# Autodesk Inventor assembly: CartesianRobotWorkSpace
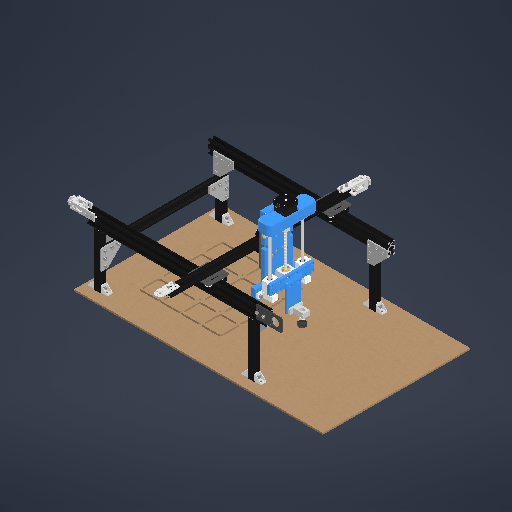
[picture p0: Inventor's stored thumbnail of the model, 512x512]
Saved by Autodesk Inventor 2027.1 (Build 311270010, 270A)
## iProperties
Created: 2026-09-29
Part Number: CartesianRobotWorkSpace
Document SubType Name: Assembly
Designer: SDS Scholar
Author: SDS Scholar
## Documents named in this file (18)
- E:\Apps\AutodeskInventor\University\MCT333_Design_of_Mechatronics_Systems_1\CAD\cartesian_robot_workspace\CartesianRobotWorkSpace.iam
- E:\Apps\AutodeskInventor\University\MCT333_Design_of_Mechatronics_Systems_1\CAD\cartesian_robot_workspace\UpperBase.ipt
- E:\Apps\AutodeskInventor\University\MCT333_Design_of_Mechatronics_Systems_1\CAD\cartesian_robot_workspace\ProductsStoringGrid.ipt
- E:\Apps\AutodeskInventor\University\MCT333_Design_of_Mechatronics_Systems_1\CAD\off_the_shelf_components\AluminiumExtrusion\AluminiumExtrusion2020\Pillars.ipt
- E:\Apps\AutodeskInventor\University\MCT333_Design_of_Mechatronics_Systems_1\CAD\off_the_shelf_components\CornerBracket2020\CornerBracket2020.ipt
- C:\Users\SDS Scholar\Documents\Inventor\Content Center Files\R2027\en-US\SS-ISO 4762\ISO 4762 - M5 x 10SS-ISO.ipt
- E:\Apps\AutodeskInventor\University\MCT333_Design_of_Mechatronics_Systems_1\CAD\off_the_shelf_components\T_nuts\Slider T-Nut for 2020 - M5.ipt
- E:\Apps\AutodeskInventor\University\MCT333_Design_of_Mechatronics_Systems_1\CAD\off_the_shelf_components\RightAngleCornerPlate2020\2020 corner joining plate v1.ipt
- E:\Apps\AutodeskInventor\University\MCT333_Design_of_Mechatronics_Systems_1\CAD\off_the_shelf_components\AluminiumExtrusion\Extrusion2040\2040extrusion_ipt\X_Axis.ipt
- E:\Apps\AutodeskInventor\University\MCT333_Design_of_Mechatronics_Systems_1\CAD\off_the_shelf_components\AluminiumExtrusion\AluminiumExtrusion2020\SupportBeam.ipt
- E:\Apps\AutodeskInventor\University\MCT333_Design_of_Mechatronics_Systems_1\CAD\off_the_shelf_components\VSoltGantrySetAllSizes\20mm Gantry Set\20mm Gantry Set.ipt
- E:\Apps\AutodeskInventor\University\MCT333_Design_of_Mechatronics_Systems_1\CAD\off_the_shelf_components\RightAngleCornerPlate2020\2020 corner joining plate v1_MIR2.ipt
- E:\Apps\AutodeskInventor\University\MCT333_Design_of_Mechatronics_Systems_1\CAD\off_the_shelf_components\T_nuts\Slider T-Nut for 2020 - M5_MIR2.ipt
- E:\Apps\AutodeskInventor\University\MCT333_Design_of_Mechatronics_Systems_1\CAD\off_the_shelf_components\nema-17-23-stepper-motor-mounts\NEMA 17 Flat.ipt
- E:\Apps\AutodeskInventor\University\MCT333_Design_of_Mechatronics_Systems_1\CAD\off_the_shelf_components\GT2BeltTensioner\2020 Belt Tensioner G_K.ipt
- E:\Apps\AutodeskInventor\University\MCT333_Design_of_Mechatronics_Systems_1\CAD\cartesian_robot_workspace\Y_Axis.iam
- E:\Apps\AutodeskInventor\University\MCT333_Design_of_Mechatronics_Systems_1\CAD\cartesian_robot_workspace\Z Axis\Z-Axis.iam
- E:\Apps\AutodeskInventor\University\MCT333_Design_of_Mechatronics_Systems_1\CAD\DESIGN1_CAD_parameters.xlsx
## Components (118 placed, 16 different names)
1. UpperBase:1 — Mate:1, Mate:2, Flush:1, Mate:4, Mate:5, Mate:6, Mate:7, Mate:8, Mate:9, Mate:10, Mate:11, Mate:12, Mate:15, Flush:2, Mate:16, Mate:17, Mate:26, Mate:27
2. ProductsStoringGrid:1 — Mate:4, Mate:5, Mate:6, Mate:7
3. ProductsStoringGrid:2 — Mate:8, Mate:9, Mate:10, Mate:11
4. Z-Axis:1 [sub-assembly] — Tangent:9, Tangent:10, Tangent:11, Tangent:12
5. SupportBeam:1 — Mate:88, Mate:123, Mate:124, Mate:125, Mate:126, Mate:138, Mate:141, Mate:143
6. X_Axis:1 — Mate:32, Mate:33, Mate:34, Mate:35, Mate:36, Mate:37, Mate:48, Mate:49, Mate:56, Mate:59, Flush:3, Mate:60, Tangent:1, Tangent:2, Tangent:3, Tangent:4, Mate:145, Mate:146, Mate:147, Mate:148, Mate:151, Mate:154, Mate:155, Flush:6, Mate:156, Mate:157, Mate:158, Mate:159, Mate:162, Mate:165, Flush:7, Mate:182
7. X_Axis:2 — Mate:89, Mate:90, Mate:91, Mate:92, Mate:93, Mate:94, Mate:107, Mate:110, Mate:113, Mate:115, Flush:4, Mate:116, Tangent:5, Tangent:6, Tangent:7, Tangent:8
8. NEMA 17 Flat:1 — Mate:149, Mate:152, Mate:155
9. Slider T-Nut for 2020 - M5:40 — Mate:145, Mate:146, Mate:150, Flush:6
10. Slider T-Nut for 2020 - M5:41 — Mate:147, Mate:148, Mate:153
11. SS ISO 4762 M5 x 10:58 — Mate:149, Mate:150, Mate:151
12. SS ISO 4762 M5 x 10:59 — Mate:152, Mate:153, Mate:154
13. 2020 Belt Tensioner G_K:1 — Mate:180, Mate:181, Mate:182
14. SS ISO 4762 M5 x 10:60 — Mate:164, Mate:165, Mate:181
15. SS ISO 4762 M5 x 10:61 — Mate:161, Mate:162, Mate:179, Mate:180
16. Slider T-Nut for 2020 - M5:42 — Mate:156, Mate:157, Mate:161, Mate:179
17. Slider T-Nut for 2020 - M5:43 — Mate:158, Mate:159, Mate:164, Flush:7
18. 20mm Gantry Set:1 — Tangent:1, Tangent:2, Tangent:3, Tangent:4, Flush:5, Mate:171, Flush:9
19. 20mm Gantry Set:2 — Tangent:5, Tangent:6, Tangent:7, Tangent:8, Flush:5, Mate:174, Mate:177, Flush:8, Flush:9
20. Y_Axis:1 [sub-assembly] — Mate:167, Mate:168, Mate:169, Mate:170, Mate:173, Mate:176, Mate:177, Flush:8, Tangent:9, Tangent:10, Tangent:11, Tangent:12
21. Slider T-Nut for 2020 - M5:44 — Mate:167, Mate:168, Mate:172
22. Slider T-Nut for 2020 - M5:45 — Mate:169, Mate:170, Mate:175
23. SS ISO 4762 M5 x 10:62 — Mate:174, Mate:175, Mate:176
24. SS ISO 4762 M5 x 10:63 — Mate:171, Mate:172, Mate:173
25. Pillars:1 — Flush:2, Mate:18, Mate:19, Mate:22, Mate:24, Mate:25, Mate:30, Mate:88, Mate:117, Mate:118, Mate:119, Mate:120, Mate:121, Mate:122, Mate:129, Mate:132, Mate:135, Mate:142, Symmetry:1
26. CornerBracket2020:4 — Mate:15, Mate:26, Mate:27, Mate:28
27. CornerBracket2020:1 — Mate:12, Mate:16, Mate:17, Mate:20, Mate:31
28. SS ISO 4762 M5 x 10:1 — Mate:20, Mate:21, Mate:22, Mate:31
29. Slider T-Nut for 2020 - M5:1 — Mate:18, Mate:19, Mate:21
30. Slider T-Nut for 2020 - M5:2 — Mate:24, Mate:25, Mate:29
31. SS ISO 4762 M5 x 10:2 — Mate:28, Mate:29, Mate:30
32. Pillars:2 — Mate:95, Mate:96, Mate:97, Mate:98, Mate:101, Mate:104, Mate:114, Mate:116
33. CornerBracket2020:5
34. CornerBracket2020:6
35. SS ISO 4762 M5 x 10:3
36. Slider T-Nut for 2020 - M5:3
37. Slider T-Nut for 2020 - M5:4
38. SS ISO 4762 M5 x 10:4
39. Pillars:3 — Symmetry:1
40. CornerBracket2020:7
41. CornerBracket2020:8
42. SS ISO 4762 M5 x 10:5
43. Slider T-Nut for 2020 - M5:5
44. Slider T-Nut for 2020 - M5:6
45. SS ISO 4762 M5 x 10:6
46. Pillars:4 — Mate:38, Mate:39, Mate:40, Mate:41, Mate:44, Mate:45, Mate:53, Mate:60
47. CornerBracket2020:9
48. CornerBracket2020:10
49. SS ISO 4762 M5 x 10:7
50. Slider T-Nut for 2020 - M5:7
51. Slider T-Nut for 2020 - M5:8
52. SS ISO 4762 M5 x 10:8
53. 2020 corner joining plate v1:6 — Mate:127, Mate:130, Mate:133, Mate:136, Mate:139, Mate:142, Mate:143, Mate:144
54. Slider T-Nut for 2020 - M5:35 — Mate:119, Mate:120, Mate:131
55. Slider T-Nut for 2020 - M5:36 — Mate:123, Mate:124, Mate:137
56. Slider T-Nut for 2020 - M5:37 — Mate:117, Mate:118, Mate:134
57. Slider T-Nut for 2020 - M5:38 — Mate:125, Mate:126, Mate:140
58. Slider T-Nut for 2020 - M5:39 — Mate:121, Mate:122, Mate:128
59. SS ISO 4762 M5 x 10:48 — Mate:127, Mate:128, Mate:129
60. SS ISO 4762 M5 x 10:49 — Mate:139, Mate:140, Mate:141
61. SS ISO 4762 M5 x 10:50 — Mate:130, Mate:131, Mate:132
62. SS ISO 4762 M5 x 10:51 — Mate:133, Mate:134, Mate:135
63. SS ISO 4762 M5 x 10:52 — Mate:136, Mate:137, Mate:138
64. 2020 corner joining plate v1_MIR2:1
65. Slider T-Nut for 2020 - M5_MIR2:1
66. Slider T-Nut for 2020 - M5_MIR2:2
67. Slider T-Nut for 2020 - M5_MIR2:3
68. Slider T-Nut for 2020 - M5_MIR2:4
69. Slider T-Nut for 2020 - M5_MIR2:5
70. SS ISO 4762 M5 x 10:53
71. SS ISO 4762 M5 x 10:54
72. SS ISO 4762 M5 x 10:55
73. SS ISO 4762 M5 x 10:56
74. SS ISO 4762 M5 x 10:57
75. 2020 corner joining plate v1:1 — Mate:42, Mate:45, Mate:46, Mate:49, Mate:51, Mate:54, Mate:57, Flush:3
76. Slider T-Nut for 2020 - M5:9 — Mate:36, Mate:37, Mate:55
77. Slider T-Nut for 2020 - M5:10 — Mate:38, Mate:39, Mate:52
78. Slider T-Nut for 2020 - M5:11 — Mate:40, Mate:41, Mate:43
79. Slider T-Nut for 2020 - M5:12 — Mate:34, Mate:35, Mate:58
80. Slider T-Nut for 2020 - M5:13 — Mate:32, Mate:33, Mate:47
81. SS ISO 4762 M5 x 10:9 — Mate:42, Mate:43, Mate:44
82. SS ISO 4762 M5 x 10:10 — Mate:46, Mate:47, Mate:48
83. SS ISO 4762 M5 x 10:11 — Mate:54, Mate:55, Mate:56
84. SS ISO 4762 M5 x 10:12 — Mate:51, Mate:52, Mate:53
85. SS ISO 4762 M5 x 10:13 — Mate:57, Mate:58, Mate:59
86. 2020 corner joining plate v1:2
87. Slider T-Nut for 2020 - M5:14
88. Slider T-Nut for 2020 - M5:15
89. Slider T-Nut for 2020 - M5:16
90. Slider T-Nut for 2020 - M5:17
91. Slider T-Nut for 2020 - M5:18
92. SS ISO 4762 M5 x 10:14
93. SS ISO 4762 M5 x 10:15
94. SS ISO 4762 M5 x 10:16
95. SS ISO 4762 M5 x 10:17
96. SS ISO 4762 M5 x 10:18
97. 2020 corner joining plate v1:4 — Mate:99, Mate:102, Mate:105, Mate:108, Mate:111, Mate:114, Mate:115, Flush:4
98. Slider T-Nut for 2020 - M5:25 — Mate:93, Mate:94, Mate:106
99. Slider T-Nut for 2020 - M5:26 — Mate:95, Mate:96, Mate:103
100. Slider T-Nut for 2020 - M5:27 — Mate:97, Mate:98, Mate:100
101. Slider T-Nut for 2020 - M5:28 — Mate:91, Mate:92, Mate:109
102. Slider T-Nut for 2020 - M5:29 — Mate:89, Mate:90, Mate:112
103. SS ISO 4762 M5 x 10:38 — Mate:99, Mate:100, Mate:101
104. SS ISO 4762 M5 x 10:39 — Mate:105, Mate:106, Mate:107
105. SS ISO 4762 M5 x 10:40 — Mate:102, Mate:103, Mate:104
106. SS ISO 4762 M5 x 10:41 — Mate:108, Mate:109, Mate:110
107. SS ISO 4762 M5 x 10:42 — Mate:111, Mate:112, Mate:113
108. 2020 corner joining plate v1:5 — Mate:144
109. Slider T-Nut for 2020 - M5:30
110. Slider T-Nut for 2020 - M5:31
111. Slider T-Nut for 2020 - M5:32
112. Slider T-Nut for 2020 - M5:33
113. Slider T-Nut for 2020 - M5:34
114. SS ISO 4762 M5 x 10:43
115. SS ISO 4762 M5 x 10:44
116. SS ISO 4762 M5 x 10:45
117. SS ISO 4762 M5 x 10:46
118. SS ISO 4762 M5 x 10:47
## Component patterns: (4 elements, first: Pillars:1 + CornerBracket2020:4 + CornerBracket2020:1 + SS ISO 4762 M5 x 10:1 + Slider T-Nut for 2020 - M5:1 + Slider T-Nut for 2020 - M5:2 + SS ISO 4762 M5 x 10:2), (2 elements, first: 2020 corner joining plate v1:6 + Slider T-Nut for 2020 - M5:35 + Slider T-Nut for 2020 - M5:36 + Slider T-Nut for 2020 - M5:37 + Slider T-Nut for 2020 - M5:38 + Slider T-Nut for 2020 - M5:39 + SS ISO 4762 M5 x 10:48 + SS ISO 4762 M5 x 10:49 + SS ISO 4762 M5 x 10:50 + SS ISO 4762 M5 x 10:51 + SS ISO 4762 M5 x 10:52), (2 elements, first: 2020 corner joining plate v1:1 + Slider T-Nut for 2020 - M5:9 + Slider T-Nut for 2020 - M5:10 + Slider T-Nut for 2020 - M5:11 + Slider T-Nut for 2020 - M5:12 + Slider T-Nut for 2020 - M5:13 + SS ISO 4762 M5 x 10:9 + SS ISO 4762 M5 x 10:10 + SS ISO 4762 M5 x 10:11 + SS ISO 4762 M5 x 10:12 + SS ISO 4762 M5 x 10:13), (2 elements, first: 2020 corner joining plate v1:4 + Slider T-Nut for 2020 - M5:25 + Slider T-Nut for 2020 - M5:26 + Slider T-Nut for 2020 - M5:27 + Slider T-Nut for 2020 - M5:28 + Slider T-Nut for 2020 - M5:29 + SS ISO 4762 M5 x 10:38 + SS ISO 4762 M5 x 10:39 + SS ISO 4762 M5 x 10:40 + SS ISO 4762 M5 x 10:41 + SS ISO 4762 M5 x 10:42)
## Relationships (168: Mate 146, Tangent 12, Flush 9, Symmetry 1)
- Mate:1: UpperBase:1
- Mate:2: UpperBase:1
- Flush:1: UpperBase:1
- Mate:4: UpperBase:1 ↔ ProductsStoringGrid:1
- Mate:5: UpperBase:1 ↔ ProductsStoringGrid:1
- Mate:6: UpperBase:1 ↔ ProductsStoringGrid:1
- Mate:7: UpperBase:1 ↔ ProductsStoringGrid:1
- Mate:8: UpperBase:1 ↔ ProductsStoringGrid:2
- Mate:9: UpperBase:1 ↔ ProductsStoringGrid:2
- Mate:10: UpperBase:1 ↔ ProductsStoringGrid:2
- Mate:11: UpperBase:1 ↔ ProductsStoringGrid:2
- Mate:12: UpperBase:1 ↔ CornerBracket2020:1
- Mate:15: UpperBase:1 ↔ CornerBracket2020:4
- Flush:2: UpperBase:1 ↔ Pillars:1
- Mate:16: UpperBase:1 ↔ CornerBracket2020:1
- Mate:17: UpperBase:1 ↔ CornerBracket2020:1
- Mate:18: Pillars:1 ↔ Slider T-Nut for 2020 - M5:1
- Mate:19: Pillars:1 ↔ Slider T-Nut for 2020 - M5:1
- Mate:20: CornerBracket2020:1 ↔ SS ISO 4762 M5 x 10:1
- Mate:21: SS ISO 4762 M5 x 10:1 ↔ Slider T-Nut for 2020 - M5:1
- Mate:22: Pillars:1 ↔ SS ISO 4762 M5 x 10:1
- Mate:24: Pillars:1 ↔ Slider T-Nut for 2020 - M5:2
- Mate:25: Pillars:1 ↔ Slider T-Nut for 2020 - M5:2
- Mate:26: UpperBase:1 ↔ CornerBracket2020:4
- Mate:27: UpperBase:1 ↔ CornerBracket2020:4
- Mate:28: CornerBracket2020:4 ↔ SS ISO 4762 M5 x 10:2
- Mate:29: Slider T-Nut for 2020 - M5:2 ↔ SS ISO 4762 M5 x 10:2
- Mate:30: Pillars:1 ↔ SS ISO 4762 M5 x 10:2
- Mate:31 (0.7 mm): CornerBracket2020:1 ↔ SS ISO 4762 M5 x 10:1
- Mate:32: X_Axis:1 ↔ Slider T-Nut for 2020 - M5:13
- Mate:33: X_Axis:1 ↔ Slider T-Nut for 2020 - M5:13
- Mate:34: X_Axis:1 ↔ Slider T-Nut for 2020 - M5:12
- Mate:35: X_Axis:1 ↔ Slider T-Nut for 2020 - M5:12
- Mate:36: X_Axis:1 ↔ Slider T-Nut for 2020 - M5:9
- Mate:37: X_Axis:1 ↔ Slider T-Nut for 2020 - M5:9
- Mate:38: Pillars:4 ↔ Slider T-Nut for 2020 - M5:10
- Mate:39: Pillars:4 ↔ Slider T-Nut for 2020 - M5:10
- Mate:40: Pillars:4 ↔ Slider T-Nut for 2020 - M5:11
- Mate:41: Pillars:4 ↔ Slider T-Nut for 2020 - M5:11
- Mate:42: 2020 corner joining plate v1:1 ↔ SS ISO 4762 M5 x 10:9
- Mate:43: Slider T-Nut for 2020 - M5:11 ↔ SS ISO 4762 M5 x 10:9
- Mate:44: Pillars:4 ↔ SS ISO 4762 M5 x 10:9
- Mate:45: Pillars:4 ↔ 2020 corner joining plate v1:1
- Mate:46: 2020 corner joining plate v1:1 ↔ SS ISO 4762 M5 x 10:10
- Mate:47: Slider T-Nut for 2020 - M5:13 ↔ SS ISO 4762 M5 x 10:10
- Mate:48: X_Axis:1 ↔ SS ISO 4762 M5 x 10:10
- Mate:49: X_Axis:1 ↔ 2020 corner joining plate v1:1
- Mate:51: 2020 corner joining plate v1:1 ↔ SS ISO 4762 M5 x 10:12
- Mate:52: Slider T-Nut for 2020 - M5:10 ↔ SS ISO 4762 M5 x 10:12
- Mate:53: Pillars:4 ↔ SS ISO 4762 M5 x 10:12
- Mate:54: 2020 corner joining plate v1:1 ↔ SS ISO 4762 M5 x 10:11
- Mate:55: Slider T-Nut for 2020 - M5:9 ↔ SS ISO 4762 M5 x 10:11
- Mate:56: X_Axis:1 ↔ SS ISO 4762 M5 x 10:11
- Mate:57: 2020 corner joining plate v1:1 ↔ SS ISO 4762 M5 x 10:13
- Mate:58: Slider T-Nut for 2020 - M5:12 ↔ SS ISO 4762 M5 x 10:13
- Mate:59: X_Axis:1 ↔ SS ISO 4762 M5 x 10:13
- Flush:3: X_Axis:1 ↔ 2020 corner joining plate v1:1
- Mate:60: X_Axis:1 ↔ Pillars:4
- Mate:88: SupportBeam:1 ↔ Pillars:1
- Tangent:1: X_Axis:1 ↔ 20mm Gantry Set:1
- Tangent:2: X_Axis:1 ↔ 20mm Gantry Set:1
- Tangent:3: X_Axis:1 ↔ 20mm Gantry Set:1
- Tangent:4: X_Axis:1 ↔ 20mm Gantry Set:1
- Mate:89: X_Axis:2 ↔ Slider T-Nut for 2020 - M5:29
- Mate:90: X_Axis:2 ↔ Slider T-Nut for 2020 - M5:29
- Mate:91: X_Axis:2 ↔ Slider T-Nut for 2020 - M5:28
- Mate:92: X_Axis:2 ↔ Slider T-Nut for 2020 - M5:28
- Mate:93: X_Axis:2 ↔ Slider T-Nut for 2020 - M5:25
- Mate:94: X_Axis:2 ↔ Slider T-Nut for 2020 - M5:25
- Mate:95: Pillars:2 ↔ Slider T-Nut for 2020 - M5:26
- Mate:96: Pillars:2 ↔ Slider T-Nut for 2020 - M5:26
- Mate:97: Pillars:2 ↔ Slider T-Nut for 2020 - M5:27
- Mate:98: Pillars:2 ↔ Slider T-Nut for 2020 - M5:27
- Mate:99: 2020 corner joining plate v1:4 ↔ SS ISO 4762 M5 x 10:38
- Mate:100: Slider T-Nut for 2020 - M5:27 ↔ SS ISO 4762 M5 x 10:38
- Mate:101: Pillars:2 ↔ SS ISO 4762 M5 x 10:38
- Mate:102: 2020 corner joining plate v1:4 ↔ SS ISO 4762 M5 x 10:40
- Mate:103: Slider T-Nut for 2020 - M5:26 ↔ SS ISO 4762 M5 x 10:40
- Mate:104: Pillars:2 ↔ SS ISO 4762 M5 x 10:40
- Mate:105: 2020 corner joining plate v1:4 ↔ SS ISO 4762 M5 x 10:39
- Mate:106: Slider T-Nut for 2020 - M5:25 ↔ SS ISO 4762 M5 x 10:39
- Mate:107: X_Axis:2 ↔ SS ISO 4762 M5 x 10:39
- Mate:108: 2020 corner joining plate v1:4 ↔ SS ISO 4762 M5 x 10:41
- Mate:109: Slider T-Nut for 2020 - M5:28 ↔ SS ISO 4762 M5 x 10:41
- Mate:110: X_Axis:2 ↔ SS ISO 4762 M5 x 10:41
- Mate:111: 2020 corner joining plate v1:4 ↔ SS ISO 4762 M5 x 10:42
- Mate:112: Slider T-Nut for 2020 - M5:29 ↔ SS ISO 4762 M5 x 10:42
- Mate:113: X_Axis:2 ↔ SS ISO 4762 M5 x 10:42
- Mate:114: Pillars:2 ↔ 2020 corner joining plate v1:4
- Mate:115: X_Axis:2 ↔ 2020 corner joining plate v1:4
- Flush:4: X_Axis:2 ↔ 2020 corner joining plate v1:4
- Mate:116: X_Axis:2 ↔ Pillars:2
- Mate:117: Pillars:1 ↔ Slider T-Nut for 2020 - M5:37
- Mate:118: Pillars:1 ↔ Slider T-Nut for 2020 - M5:37
- Mate:119: Pillars:1 ↔ Slider T-Nut for 2020 - M5:35
- Mate:120: Pillars:1 ↔ Slider T-Nut for 2020 - M5:35
- Mate:121: Pillars:1 ↔ Slider T-Nut for 2020 - M5:39
- Mate:122: Pillars:1 ↔ Slider T-Nut for 2020 - M5:39
- Mate:123: SupportBeam:1 ↔ Slider T-Nut for 2020 - M5:36
- Mate:124: SupportBeam:1 ↔ Slider T-Nut for 2020 - M5:36
- Mate:125: SupportBeam:1 ↔ Slider T-Nut for 2020 - M5:38
- Mate:126: SupportBeam:1 ↔ Slider T-Nut for 2020 - M5:38
- Mate:127: 2020 corner joining plate v1:6 ↔ SS ISO 4762 M5 x 10:48
- Mate:128: Slider T-Nut for 2020 - M5:39 ↔ SS ISO 4762 M5 x 10:48
- Mate:129: Pillars:1 ↔ SS ISO 4762 M5 x 10:48
- Mate:130: 2020 corner joining plate v1:6 ↔ SS ISO 4762 M5 x 10:50
- Mate:131: Slider T-Nut for 2020 - M5:35 ↔ SS ISO 4762 M5 x 10:50
- Mate:132: Pillars:1 ↔ SS ISO 4762 M5 x 10:50
- Mate:133: 2020 corner joining plate v1:6 ↔ SS ISO 4762 M5 x 10:51
- Mate:134: Slider T-Nut for 2020 - M5:37 ↔ SS ISO 4762 M5 x 10:51
- Mate:135: Pillars:1 ↔ SS ISO 4762 M5 x 10:51
- Mate:136: 2020 corner joining plate v1:6 ↔ SS ISO 4762 M5 x 10:52
- Mate:137: Slider T-Nut for 2020 - M5:36 ↔ SS ISO 4762 M5 x 10:52
- Mate:138: SupportBeam:1 ↔ SS ISO 4762 M5 x 10:52
- Mate:139: 2020 corner joining plate v1:6 ↔ SS ISO 4762 M5 x 10:49
- Mate:140: Slider T-Nut for 2020 - M5:38 ↔ SS ISO 4762 M5 x 10:49
- Mate:141: SupportBeam:1 ↔ SS ISO 4762 M5 x 10:49
- Mate:142: Pillars:1 ↔ 2020 corner joining plate v1:6
- Mate:143: SupportBeam:1 ↔ 2020 corner joining plate v1:6
- Symmetry:1: Pillars:1 ↔ Pillars:3
- Mate:144 (5 mm): 2020 corner joining plate v1:6 ↔ 2020 corner joining plate v1:5
- Tangent:5: X_Axis:2 ↔ 20mm Gantry Set:2
- Tangent:6: X_Axis:2 ↔ 20mm Gantry Set:2
- Tangent:7: X_Axis:2 ↔ 20mm Gantry Set:2
- Tangent:8: X_Axis:2 ↔ 20mm Gantry Set:2
- Flush:5: 20mm Gantry Set:1 ↔ 20mm Gantry Set:2
- Mate:145: X_Axis:1 ↔ Slider T-Nut for 2020 - M5:40
- Mate:146: X_Axis:1 ↔ Slider T-Nut for 2020 - M5:40
- Mate:147: X_Axis:1 ↔ Slider T-Nut for 2020 - M5:41
- Mate:148: X_Axis:1 ↔ Slider T-Nut for 2020 - M5:41
- Mate:149: NEMA 17 Flat:1 ↔ SS ISO 4762 M5 x 10:58
- Mate:150: Slider T-Nut for 2020 - M5:40 ↔ SS ISO 4762 M5 x 10:58
- Mate:151: X_Axis:1 ↔ SS ISO 4762 M5 x 10:58
- Mate:152: NEMA 17 Flat:1 ↔ SS ISO 4762 M5 x 10:59
- Mate:153: Slider T-Nut for 2020 - M5:41 ↔ SS ISO 4762 M5 x 10:59
- Mate:154: X_Axis:1 ↔ SS ISO 4762 M5 x 10:59
- Mate:155: X_Axis:1 ↔ NEMA 17 Flat:1
- Flush:6: X_Axis:1 ↔ Slider T-Nut for 2020 - M5:40
- Mate:156: X_Axis:1 ↔ Slider T-Nut for 2020 - M5:42
- Mate:157: X_Axis:1 ↔ Slider T-Nut for 2020 - M5:42
- Mate:158: X_Axis:1 ↔ Slider T-Nut for 2020 - M5:43
- Mate:159: X_Axis:1 ↔ Slider T-Nut for 2020 - M5:43
- Mate:161: SS ISO 4762 M5 x 10:61 ↔ Slider T-Nut for 2020 - M5:42
- Mate:162: X_Axis:1 ↔ SS ISO 4762 M5 x 10:61
- Mate:164: SS ISO 4762 M5 x 10:60 ↔ Slider T-Nut for 2020 - M5:43
- Mate:165: X_Axis:1 ↔ SS ISO 4762 M5 x 10:60
- Flush:7: X_Axis:1 ↔ Slider T-Nut for 2020 - M5:43
- Mate:167: Y_Axis:1 ↔ Slider T-Nut for 2020 - M5:44
- Mate:168: Y_Axis:1 ↔ Slider T-Nut for 2020 - M5:44
- Mate:169: Y_Axis:1 ↔ Slider T-Nut for 2020 - M5:45
- Mate:170: Y_Axis:1 ↔ Slider T-Nut for 2020 - M5:45
- Mate:171: 20mm Gantry Set:1 ↔ SS ISO 4762 M5 x 10:63
- Mate:172: Slider T-Nut for 2020 - M5:44 ↔ SS ISO 4762 M5 x 10:63
- Mate:173: Y_Axis:1 ↔ SS ISO 4762 M5 x 10:63
- Mate:174: 20mm Gantry Set:2 ↔ SS ISO 4762 M5 x 10:62
- Mate:175: Slider T-Nut for 2020 - M5:45 ↔ SS ISO 4762 M5 x 10:62
- Mate:176: Y_Axis:1 ↔ SS ISO 4762 M5 x 10:62
- Mate:177: 20mm Gantry Set:2 ↔ Y_Axis:1
- Flush:8 (-20 mm): 20mm Gantry Set:2 ↔ Y_Axis:1
- Flush:9: 20mm Gantry Set:1 ↔ 20mm Gantry Set:2
- Mate:179: SS ISO 4762 M5 x 10:61 ↔ Slider T-Nut for 2020 - M5:42
- Mate:180: 2020 Belt Tensioner G_K:1 ↔ SS ISO 4762 M5 x 10:61
- Mate:181: 2020 Belt Tensioner G_K:1 ↔ SS ISO 4762 M5 x 10:60
- Mate:182: X_Axis:1 ↔ 2020 Belt Tensioner G_K:1
- Tangent:9: Z-Axis:1 ↔ Y_Axis:1
- Tangent:10: Z-Axis:1 ↔ Y_Axis:1
- Tangent:11: Z-Axis:1 ↔ Y_Axis:1
- Tangent:12: Z-Axis:1 ↔ Y_Axis:1
## Named parameters: Product_dia = 50 mm, ProductBaseHeight = 40 mm, ProductLedHeight = 20 mm, GridProcutClearance = 3 mm, GridBorderThickness = 5 mm, GridBorderFillets = 7 mm, GridTotalSize = 63 mm, GridRobotClearance = 50 mm, AluminiumExtrusionBase = 20 mm, AluminiumExtrusionClearance = 30 mm, BaseTotalWidth = 452 mm, FeedingAreaLength = 600 mm, BaseTotalLength = 764 mm, DistanceBetweenGrid = 5 mm, WorkspaceLength = 552 mm, WorkspaceWidth = 372 mm, WorkspaceHeight = 168.5 mm, AxesBaseFillet = 15 mm, Zaxis = 127 mm, ProductTotalHeight = 45 mm, VerticalClearance = 10 mm, VerticalStroke = 85 mm, FrontArea = 150 mm, BackArea = 50 mm
